# Autodesk Inventor assembly: Shoulder_
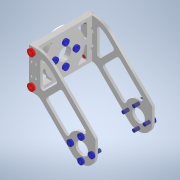
[picture p0: Inventor's stored thumbnail of the model, 180x180]
Saved by Autodesk Inventor 2020.4 (Build 244396000, 396)
## iProperties
Created: 2022-01-10
Part Number: Shoulder_
Document SubType Name: Assembly
Designer: Masato Kubotera
Author: Masato Kubotera
## Documents named in this file (7)
- C:\Users\Masato\Documents\Inventor\CIT Brains_Inventor\OpenPlatform_ver3_0 - ve4_1 branch\UpperBody\Arm\Shoulder_.iam
- C:\Users\Masato\Documents\Inventor\CIT Brains_Inventor\OpenPlatform_ver3_0 - ve4_1 branch\Ready_Made\TT-2532-10.ipt
- C:\Users\Masato\Documents\Inventor\CIT Brains_Inventor\OpenPlatform_ver3_0 - ve4_1 branch\UpperBody\Arm\Shoulder_horn_frame.ipt
- C:\Users\Masato\Documents\Inventor\CIT Brains_Inventor\OpenPlatform_ver3_0 - ve4_1 branch\UpperBody\Arm\Shoulder_side_frame_.ipt
- C:\Users\Masato\Documents\Inventor\CIT Brains_Inventor\OpenPlatform_ver3_0 - ve4_1 branch\Ready_Made\Screw\M2_6-6.ipt
- C:\Users\Masato\Documents\Inventor\CIT Brains_Inventor\OpenPlatform_ver3_0 - ve4_1 branch\Ready_Made\Screw\M2_6-8.ipt
- C:\Users\Masato\Documents\Inventor\CIT Brains_Inventor\OpenPlatform_ver3_0 - ve4_1 branch\Ready_Made\Screw\M3-6.ipt
## Components (20 placed, 6 different names)
1. TT-2532-10:1 — 挿入:1
2. Shoulder_horn_frame:1 — メイト:1, メイト:2, メイト:3, 挿入:1, 挿入:2, 挿入:3, 挿入:4, 挿入:5, 挿入:14, 挿入:15, 挿入:16, 挿入:17
3. Shoulder_side_frame_:1 — 挿入:2, 挿入:3, 挿入:6, 挿入:7, 挿入:8, 挿入:9, 挿入:18, 挿入:19
4. Shoulder_side_frame_:2 — 挿入:4, 挿入:5, 挿入:10, 挿入:11, 挿入:12, 挿入:13, 挿入:20, 挿入:21
5. M2_6-6:1 — 挿入:6
6. M2_6-6:2 — 挿入:7
7. M2_6-6:3 — 挿入:8
8. M2_6-6:4 — 挿入:9
9. M2_6-6:5 — 挿入:10
10. M2_6-6:6 — 挿入:11
11. M2_6-6:7 — 挿入:12
12. M2_6-6:8 — 挿入:13
13. M2_6-8:1 — 挿入:14
14. M2_6-8:2 — 挿入:15
15. M2_6-8:3 — 挿入:16
16. M2_6-8:4 — 挿入:17
17. M3-6:1 — 挿入:18
18. M3-6:2 — 挿入:19
19. M3-6:3 — 挿入:20
20. M3-6:4 — 挿入:21
## Relationships (24: Insert 21, Mate 3)
- メイト:1 [Mate]: Shoulder_horn_frame:1
- メイト:2 [Mate]: Shoulder_horn_frame:1
- メイト:3 [Mate]: Shoulder_horn_frame:1
- 挿入:1 [Insert]: TT-2532-10:1 ↔ Shoulder_horn_frame:1
- 挿入:2 [Insert]: Shoulder_horn_frame:1 ↔ Shoulder_side_frame_:1
- 挿入:3 [Insert]: Shoulder_horn_frame:1 ↔ Shoulder_side_frame_:1
- 挿入:4 [Insert]: Shoulder_horn_frame:1 ↔ Shoulder_side_frame_:2
- 挿入:5 [Insert]: Shoulder_horn_frame:1 ↔ Shoulder_side_frame_:2
- 挿入:6 [Insert]: Shoulder_side_frame_:1 ↔ M2_6-6:1
- 挿入:7 [Insert]: Shoulder_side_frame_:1 ↔ M2_6-6:2
- 挿入:8 [Insert]: Shoulder_side_frame_:1 ↔ M2_6-6:3
- 挿入:9 [Insert]: Shoulder_side_frame_:1 ↔ M2_6-6:4
- 挿入:10 [Insert]: Shoulder_side_frame_:2 ↔ M2_6-6:5
- 挿入:11 [Insert]: Shoulder_side_frame_:2 ↔ M2_6-6:6
- 挿入:12 [Insert]: Shoulder_side_frame_:2 ↔ M2_6-6:7
- 挿入:13 [Insert]: Shoulder_side_frame_:2 ↔ M2_6-6:8
- 挿入:14 [Insert]: Shoulder_horn_frame:1 ↔ M2_6-8:1
- 挿入:15 [Insert]: Shoulder_horn_frame:1 ↔ M2_6-8:2
- 挿入:16 [Insert]: Shoulder_horn_frame:1 ↔ M2_6-8:3
- 挿入:17 [Insert]: Shoulder_horn_frame:1 ↔ M2_6-8:4
- 挿入:18 [Insert]: Shoulder_side_frame_:1 ↔ M3-6:1
- 挿入:19 [Insert]: Shoulder_side_frame_:1 ↔ M3-6:2
- 挿入:20 [Insert]: Shoulder_side_frame_:2 ↔ M3-6:3
- 挿入:21 [Insert]: Shoulder_side_frame_:2 ↔ M3-6:4
